# Autodesk Inventor assembly: roller cage_MIR
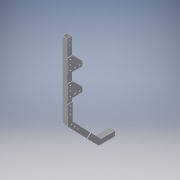
[picture p0: Inventor's stored thumbnail of the model, 180x180]
Saved by Autodesk Inventor 2016 (Build 200138000, 138)
## iProperties
Created: 2016-02-02
Part Number: roller cage_MIR
Document SubType Name: Assembly
Designer: gus
Mass: 261.186 g
Surface Area: 977.44 cm^2
Volume: 96.7354 cm^3
Density: 2.7 g/cm^3
Author: gus
## Documents named in this file (8)
- \\Mac\Home\Desktop\1510-stronghold-CAD-master\roller cage\roller cage_MIR.iam
- \\Mac\Home\Desktop\1510-stronghold-CAD-master\roller cage\top_MIR.ipt
- \\Mac\Home\Desktop\1510-stronghold-CAD-master\roller cage\gusset plate_MIR.ipt
- \\Mac\Home\Desktop\1510-stronghold-CAD-master\roller cage\robot_MIR.iam
- \\Mac\Home\Desktop\1510-stronghold-CAD-master\roller cage\frontrollcage.ipt
- \\Mac\Home\Desktop\1510-stronghold-CAD-master\roller cage\front support.ipt
- \\Mac\Home\Desktop\1510-stronghold-CAD-master\roller cage\lower gusset.ipt
- \\Mac\Home\Desktop\1510-stronghold-CAD-master\roller cage\bottom gusset.ipt
## Components (8 placed, 7 different names)
1. top_MIR:1 — Mate:8, Mate:7, Mate:3, Mate:11, Mate:10, Mate:9, Mate:10, Flush:1, Mate:13, Flush:3
2. gusset plate_MIR:1 — Mate:8, Mate:7, Mate:3
3. gusset plate_MIR:2 — Mate:11, Mate:10, Mate:9
4. frontrollcage:1 — Mate:10, Flush:1, Flush:2, Mate:11, Mate:12, Flush:4, Mate:14, Flush:6
5. robot_MIR:1 [sub-assembly]
6. front support:1 — Flush:2, Mate:11, Mate:12, Flush:5
7. lower gusset:1 — Mate:13, Flush:3, Flush:4
8. bottom gusset:1 — Mate:14, Flush:5, Flush:6
## Relationships (17: Mate 11, Flush 6)
- Mate:8: top_MIR:1 ↔ gusset plate_MIR:1
- Mate:7: top_MIR:1 ↔ gusset plate_MIR:1
- Mate:3: top_MIR:1 ↔ gusset plate_MIR:1
- Mate:11: top_MIR:1 ↔ gusset plate_MIR:2
- Mate:10: top_MIR:1 ↔ gusset plate_MIR:2
- Mate:9: top_MIR:1 ↔ gusset plate_MIR:2
- Mate:10: top_MIR:1 ↔ frontrollcage:1
- Flush:1: top_MIR:1 ↔ frontrollcage:1
- Flush:2: frontrollcage:1 ↔ front support:1
- Mate:11: frontrollcage:1 ↔ front support:1
- Mate:12: frontrollcage:1 ↔ front support:1
- Mate:13: top_MIR:1 ↔ lower gusset:1
- Flush:3: top_MIR:1 ↔ lower gusset:1
- Flush:4: frontrollcage:1 ↔ lower gusset:1
- Mate:14: frontrollcage:1 ↔ bottom gusset:1
- Flush:5: front support:1 ↔ bottom gusset:1
- Flush:6: frontrollcage:1 ↔ bottom gusset:1
